# Autodesk Inventor assembly: Telemetry TAZ V1_Simplify_1
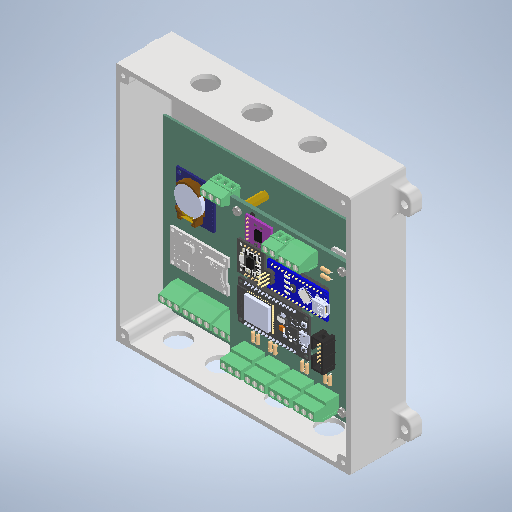
[picture p0: Inventor's stored thumbnail of the model, 512x512]
Saved by Autodesk Inventor 2025.2 (Build 292293000, 293)
## iProperties
Created: 2025-02-25
Part Number: Telemetry TAZ V1_Simplify_1
Document SubType Name: Assembly
Designer: nugro
Author: nugro
## Documents named in this file (3)
- C:\Users\nugro\Documents\KiCad\Telemetry TAZ V1\Telemetry TAZ V1\Telemetry TAZ V1\Telemetry TAZ V1\Telemetry TAZ V1_Simplify_1.iam
- C:\Users\nugro\Documents\KiCad\Telemetry TAZ V1\Telemetry TAZ V1\Telemetry TAZ V1\Telemetry TAZ V1\Solid1.ipt
- C:\Users\nugro\Documents\KiCad\boxpcb new 4 rev\boxpcb new 4 rev\boxpcb new 4 rev.ipt
## Components (2 placed, 2 different names)
1. Solid1:1 — Mate:1
2. boxpcb new 4 rev:1 — Mate:1
## Relationships (1: Mate 1)
- Mate:1: Solid1:1 ↔ boxpcb new 4 rev:1
